# Autodesk Inventor assembly: Ensamblaje1
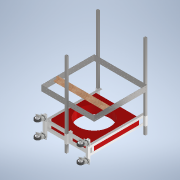
[picture p0: Inventor's stored thumbnail of the model, 180x180]
Saved by Autodesk Inventor 2020 (Build 240168000, 168)
## iProperties
Created: 2022-03-23
Part Number: Ensamblaje1
Document SubType Name: Assembly
Designer: aarco
Author: aarco
## Documents named in this file (7)
- C:\Users\aarco\Desktop\IDOM\REV_2\Ensamblaje1.iam
- C:\Users\aarco\Desktop\IDOM\REV_2\Latch.ipt
- C:\Users\aarco\Desktop\IDOM\REV_2\SoporteBobina.ipt
- C:\Users\aarco\Desktop\IDOM\REV_2\Madera.ipt
- C:\Users\aarco\Desktop\IDOM\REV_2\Bobina.ipt
- C:\Users\aarco\Desktop\IDOM\REV_2\Grid.ipt
- C:\Users\aarco\Desktop\IDOM\REV_2\BPAB 1001 6150.ipt
## Components (12 placed, 6 different names)
1. Latch:1 — Rígido:1
2. SoporteBobina:1 — Coincidencia:1, Coincidencia:3, Coincidencia:4, Nivelación:1, Coincidencia:7, Coincidencia:18, Coincidencia:19, Nivelación:9, Nivelación:10
3. Madera:1 — Rígido:1, Rígido:2, Coincidencia:13, Ángulo:1, Rígido:3, Rígido:4, Coincidencia:14, Coincidencia:15, Nivelación:8
4. Latch:2 — Rígido:2
5. Bobina:1 — Coincidencia:1, Coincidencia:3, Coincidencia:4
6. Grid:1 — Coincidencia:14, Coincidencia:15, Nivelación:8, Coincidencia:17, Coincidencia:18
7. Latch:3 — Rígido:3
8. Latch:4 — Rígido:4
9. BPAB 1001 6150:1 — Coincidencia:19, Nivelación:9, Nivelación:10
10. BPAB 1001 6150:2
11. BPAB 1001 6150:3
12. BPAB 1001 6150:4
## Component patterns: (4 elements, first: BPAB 1001 6150:1)
## Relationships (19: Mate 10, WeldJoint 4, Flush 4, Angle 1)
- Rígido:1 [WeldJoint]: Latch:1 ↔ Madera:1
- Rígido:2 [WeldJoint]: Madera:1 ↔ Latch:2
- Coincidencia:1 [Mate]: SoporteBobina:1 ↔ Bobina:1
- Coincidencia:3 [Mate]: SoporteBobina:1 ↔ Bobina:1
- Coincidencia:4 [Mate]: SoporteBobina:1 ↔ Bobina:1
- Nivelación:1 [Flush] (500 mm): SoporteBobina:1
- Coincidencia:7 [Mate]: SoporteBobina:1
- Coincidencia:13 [Mate]: Madera:1
- Ángulo:1 [Angle] (0 deg): Madera:1
- Rígido:3 [WeldJoint]: Madera:1 ↔ Latch:3
- Rígido:4 [WeldJoint]: Madera:1 ↔ Latch:4
- Coincidencia:14 [Mate]: Madera:1 ↔ Grid:1
- Coincidencia:15 [Mate] (400 mm): Madera:1 ↔ Grid:1
- Nivelación:8 [Flush]: Madera:1 ↔ Grid:1
- Coincidencia:17 [Mate]: Grid:1
- Coincidencia:18 [Mate] (800 mm): SoporteBobina:1 ↔ Grid:1
- Coincidencia:19 [Mate]: SoporteBobina:1 ↔ BPAB 1001 6150:1
- Nivelación:9 [Flush] (-2.5 mm): SoporteBobina:1 ↔ BPAB 1001 6150:1
- Nivelación:10 [Flush] (-2.5 mm): SoporteBobina:1 ↔ BPAB 1001 6150:1
